# Autodesk Inventor assembly: 276-2193
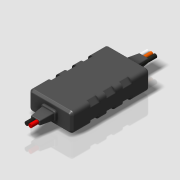
[picture p0: Inventor's stored thumbnail of the model, 180x180]
Saved by Autodesk Inventor 2015 SP1 (Build 190201100, 201)
## iProperties
Category: Motion
Company: Super Sonic Sparks, Team 24
Document SubType Name: Assembly
Designer: Jordan Kiesel
Catalog Web Link: vexrobotics.com/276-2193.html
Vendor: VEX Robotics, Inc.
Part Number: 276-2193
Description: Uses a standard PWM signal to drive a VEX 2-Wire Motor.
Mass: 9.19351 g
Surface Area: 31.0048 cm^2
Volume: 5.53592 cm^3
Density: 1.6607 g/cm^3
Translation Standard: STEP AP214IS
FileName: Motor Controller 29.iam
PreProcessor: Autodesk Inventor 2012
PostProcessor: Build: 138, Release: 2013 RTM - Date: Thu 03/01/2012
Sent Units: inch
Uncertainty: 0.00039370078740199997
Author: Jordan Kiesel
Title: Motor Controller 29
Comments: The VEX Motor Controller 29 uses a standard PWM signal (like that originating from the 3-wire ports on VEX Microcontrollers) to drive a VEX 2-Wire Motor. Note: We recommend using no more more than one (1) 3-Wire extension cable in between the Motor Controller 29 and a VEX Microcontroller. For longer extensions, use 2-Wire extension cables in between the Motor Controller 29 and a VEX 2-Wire motor.
## Documents named in this file (6)
- C:\Users\Jordan\Documents\Robotics\VEX\CAD\2015 BNS CAD Library (beta)\Motion\Motors\Motor Controller 29.iam
- C:\Users\Jordan\Documents\Robotics\VEX\CAD\2015 BNS CAD Library (beta)\Motion\Motors\Reference Parts\Motor Controller 29\Motor Controller.ipt
- C:\Users\Jordan\Documents\Robotics\VEX\CAD\2015 BNS CAD Library (beta)\Motion\Motors\Reference Parts\Motors\3-Wire Cable Support.ipt
- C:\Users\Jordan\Documents\Robotics\VEX\CAD\2015 BNS CAD Library (beta)\Motion\Motors\Reference Parts\Motors\2-Wire Cable Support.ipt
- C:\Users\Jordan\Documents\Robotics\VEX\CAD\2015 BNS CAD Library (beta)\Motion\Motors\Reference Parts\Motor Controller 29\2-Wire Cable, Cut.ipt
- C:\Users\Jordan\Documents\Robotics\VEX\CAD\2015 BNS CAD Library (beta)\Motion\Motors\Reference Parts\Motors\3-Wire Black-Orange-White Cable, Cut.ipt
## Components (5 placed, 5 different names)
1. Motor Controller:1
2. 2-Wire Cable Support:1 — Angle:1, Tangent:1, Tangent:2, Tangent:3
3. 3-Wire Cable Support:1 — Angle:2, Tangent:4, Tangent:5, Tangent:6
4. 2-Wire Cable, Cut:1 — Angle:1, Tangent:1, Tangent:2, Tangent:3
5. 3-Wire Black-Orange-White Cable, Cut:1 — Angle:2, Tangent:4, Tangent:5, Tangent:6
## Relationships (8: Tangent 6, Angle 2)
- Angle:1 (0 deg): 2-Wire Cable Support:1 ↔ 2-Wire Cable, Cut:1
- Tangent:1 (0.2286 mm): 2-Wire Cable Support:1 ↔ 2-Wire Cable, Cut:1
- Tangent:2 (0.2286 mm): 2-Wire Cable Support:1 ↔ 2-Wire Cable, Cut:1
- Tangent:3 (0.1397 mm): 2-Wire Cable Support:1 ↔ 2-Wire Cable, Cut:1
- Angle:2 (0 deg): 3-Wire Cable Support:1 ↔ 3-Wire Black-Orange-White Cable, Cut:1
- Tangent:4 (0.2286 mm): 3-Wire Cable Support:1 ↔ 3-Wire Black-Orange-White Cable, Cut:1
- Tangent:5 (0.2286 mm): 3-Wire Cable Support:1 ↔ 3-Wire Black-Orange-White Cable, Cut:1
- Tangent:6 (1.2319 mm): 3-Wire Cable Support:1 ↔ 3-Wire Black-Orange-White Cable, Cut:1
